# Autodesk Inventor assembly: KeyPrinting
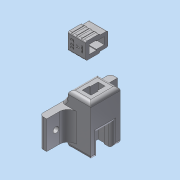
[picture p0: Inventor's stored thumbnail of the model, 180x180]
Saved by Autodesk Inventor 2015 SP1 (Build 190203100, 203)
## iProperties
Created: 2015-07-03
Part Number: KeyPrinting
Document SubType Name: Assembly
Designer: YOUR_NAME_HERE
Author: YOUR_NAME_HERE
## Documents named in this file (3)
- C:\Users\Rahul\Electric Skateboard\Electric Skateboard CAD\KeyPrinting.iam
- C:\Users\Rahul\Electric Skateboard\Electric Skateboard CAD\ArmingKeySlot.ipt
- C:\Users\Rahul\Electric Skateboard\Electric Skateboard CAD\ArmingKey.ipt
## Components (2 placed, 2 different names)
1. ArmingKeySlot:1 — Flush:1, Flush:2, Mate:1
2. ArmingKey:1 — Flush:1, Flush:2, Mate:1
## Relationships (3: Flush 2, Mate 1)
- Flush:1: ArmingKeySlot:1 ↔ ArmingKey:1
- Flush:2: ArmingKeySlot:1 ↔ ArmingKey:1
- Mate:1 (25.4 mm): ArmingKeySlot:1 ↔ ArmingKey:1
